# Autodesk Inventor assembly: A2017_T2_01
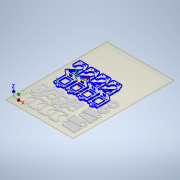
[picture p0: Inventor's stored thumbnail of the model, 180x180]
Saved by Autodesk Inventor 2020 (Build 240168000, 168)
## iProperties
Created: 2021-08-27
Part Number: A2017_T2_01
Document SubType Name: Assembly
Designer: Masato
Author: Masato
## Documents named in this file (8)
- D:\GitHub\inventor\SUSTAINA-OP\Cam\A2017_T2_01.iam
- D:\GitHub\inventor\SUSTAINA-OP\Cam\DisposableBoard.ipt
- D:\GitHub\inventor\SUSTAINA-OP\LowerBody\Ankle\Ankle_back_frame.ipt
- D:\GitHub\inventor\SUSTAINA-OP\LowerBody\Foot\Foot_back_frame.ipt
- D:\GitHub\inventor\SUSTAINA-OP\LowerBody\Foot\Foot_front_frame.ipt
- D:\GitHub\inventor\SUSTAINA-OP\LowerBody\Leg_joit\Leg_joint_pitch_frame.ipt
- D:\GitHub\inventor\SUSTAINA-OP\LowerBody\Ankle\Ankle_side_frame.ipt
- D:\GitHub\inventor\SUSTAINA-OP\UpperBody\Trunk\CrossRollerBearing\Inner_flange.ipt
## Components (19 placed, 7 different names)
1. DisposableBoard:1 — メイト:2, メイト:1, フラッシュ:1, フラッシュ:2, メイト:4, メイト:5, メイト:6, メイト:7, メイト:9, メイト:10, メイト:11, メイト:12, メイト:13, メイト:17, メイト:18, メイト:19, メイト:20, メイト:21, メイト:22, メイト:23, 正接:1, 正接:3, メイト:26, メイト:27, メイト:29, メイト:31, メイト:34, メイト:36, メイト:37, メイト:38, メイト:41, メイト:43, メイト:46, メイト:47, 角度:1, 角度:2
2. Ankle_back_frame:1 — メイト:4, メイト:9, メイト:10, メイト:14, メイト:28, 正接:4
3. Ankle_back_frame:2 — メイト:5, メイト:11, メイト:14, メイト:15
4. Ankle_back_frame:3 — メイト:6, メイト:12, メイト:15, メイト:16, メイト:33, 正接:5
5. Ankle_back_frame:4 — メイト:7, メイト:13, メイト:16
6. Foot_back_frame:2 — メイト:19, メイト:22, メイト:23, メイト:24
7. Foot_front_frame:1 — メイト:17, メイト:21, 正接:2, メイト:25
8. Foot_front_frame:2 — メイト:18, メイト:25, 正接:3, メイト:45, 正接:9
9. Foot_back_frame:3 — メイト:20, 正接:1, メイト:24, 正接:2
10. Leg_joint_pitch_frame:1 — メイト:26, メイト:27, メイト:28, メイト:30, 正接:6
11. Leg_joint_pitch_frame:2 — メイト:31, メイト:32, メイト:33, メイト:35, 正接:7
12. Leg_joint_pitch_frame:3 — メイト:29, メイト:30, 正接:4, メイト:32, メイト:39
13. Leg_joint_pitch_frame:4 — メイト:34, メイト:35, 正接:5
14. Ankle_side_frame:1 — メイト:36, メイト:37, 正接:6, メイト:40
15. Ankle_side_frame:2 — メイト:38, メイト:39, メイト:40, メイト:42
16. Ankle_side_frame:3 — メイト:41, メイト:42, 正接:7, メイト:44
17. Ankle_side_frame:4 — メイト:43, メイト:44, メイト:45, 正接:8, 正接:11
18. Inner_flange:1 — メイト:46, 角度:1, 正接:8, 正接:9, 正接:10
19. Inner_flange:2 — メイト:47, 正接:10, 正接:11, 角度:2
## Relationships (60: Mate 45, Tangent 11, Flush 2, Angle 2)
- メイト:2 [Mate]: DisposableBoard:1
- メイト:1 [Mate]: DisposableBoard:1
- フラッシュ:1 [Flush]: DisposableBoard:1
- フラッシュ:2 [Flush]: DisposableBoard:1
- メイト:4 [Mate]: DisposableBoard:1 ↔ Ankle_back_frame:1
- メイト:5 [Mate]: DisposableBoard:1 ↔ Ankle_back_frame:2
- メイト:6 [Mate]: DisposableBoard:1 ↔ Ankle_back_frame:3
- メイト:7 [Mate]: DisposableBoard:1 ↔ Ankle_back_frame:4
- メイト:9 [Mate] (3 mm): DisposableBoard:1 ↔ Ankle_back_frame:1
- メイト:10 [Mate] (3 mm): DisposableBoard:1 ↔ Ankle_back_frame:1
- メイト:11 [Mate] (3 mm): DisposableBoard:1 ↔ Ankle_back_frame:2
- メイト:12 [Mate] (3 mm): DisposableBoard:1 ↔ Ankle_back_frame:3
- メイト:13 [Mate] (3 mm): DisposableBoard:1 ↔ Ankle_back_frame:4
- メイト:14 [Mate] (2.5 mm): Ankle_back_frame:1 ↔ Ankle_back_frame:2
- メイト:15 [Mate] (2.5 mm): Ankle_back_frame:2 ↔ Ankle_back_frame:3
- メイト:16 [Mate] (2.5 mm): Ankle_back_frame:3 ↔ Ankle_back_frame:4
- メイト:17 [Mate]: DisposableBoard:1 ↔ Foot_front_frame:1
- メイト:18 [Mate]: DisposableBoard:1 ↔ Foot_front_frame:2
- メイト:19 [Mate]: DisposableBoard:1 ↔ Foot_back_frame:2
- メイト:20 [Mate]: DisposableBoard:1 ↔ Foot_back_frame:3
- メイト:21 [Mate] (3 mm): DisposableBoard:1 ↔ Foot_front_frame:1
- メイト:22 [Mate] (3 mm): DisposableBoard:1 ↔ Foot_back_frame:2
- メイト:23 [Mate] (3 mm): DisposableBoard:1 ↔ Foot_back_frame:2
- 正接:1 [Tangent] (3 mm): DisposableBoard:1 ↔ Foot_back_frame:3
- メイト:24 [Mate] (2.5 mm): Foot_back_frame:2 ↔ Foot_back_frame:3
- 正接:2 [Tangent] (2.5 mm): Foot_front_frame:1 ↔ Foot_back_frame:3
- メイト:25 [Mate] (2.5 mm): Foot_front_frame:1 ↔ Foot_front_frame:2
- 正接:3 [Tangent] (3 mm): DisposableBoard:1 ↔ Foot_front_frame:2
- メイト:26 [Mate]: DisposableBoard:1 ↔ Leg_joint_pitch_frame:1
- メイト:27 [Mate] (3 mm): DisposableBoard:1 ↔ Leg_joint_pitch_frame:1
- メイト:28 [Mate] (2.5 mm): Ankle_back_frame:1 ↔ Leg_joint_pitch_frame:1
- メイト:29 [Mate]: DisposableBoard:1 ↔ Leg_joint_pitch_frame:3
- メイト:30 [Mate] (2.5 mm): Leg_joint_pitch_frame:1 ↔ Leg_joint_pitch_frame:3
- 正接:4 [Tangent] (2.5 mm): Ankle_back_frame:1 ↔ Leg_joint_pitch_frame:3
- メイト:31 [Mate]: DisposableBoard:1 ↔ Leg_joint_pitch_frame:2
- メイト:32 [Mate] (2.5 mm): Leg_joint_pitch_frame:2 ↔ Leg_joint_pitch_frame:3
- メイト:33 [Mate] (2.5 mm): Ankle_back_frame:3 ↔ Leg_joint_pitch_frame:2
- メイト:34 [Mate]: DisposableBoard:1 ↔ Leg_joint_pitch_frame:4
- メイト:35 [Mate] (2.5 mm): Leg_joint_pitch_frame:2 ↔ Leg_joint_pitch_frame:4
- 正接:5 [Tangent] (2.5 mm): Ankle_back_frame:3 ↔ Leg_joint_pitch_frame:4
- メイト:36 [Mate]: DisposableBoard:1 ↔ Ankle_side_frame:1
- メイト:37 [Mate] (3 mm): DisposableBoard:1 ↔ Ankle_side_frame:1
- 正接:6 [Tangent] (2.5 mm): Leg_joint_pitch_frame:1 ↔ Ankle_side_frame:1
- メイト:38 [Mate]: DisposableBoard:1 ↔ Ankle_side_frame:2
- メイト:39 [Mate] (2.5 mm): Leg_joint_pitch_frame:3 ↔ Ankle_side_frame:2
- メイト:40 [Mate] (2.5 mm): Ankle_side_frame:1 ↔ Ankle_side_frame:2
- メイト:41 [Mate]: DisposableBoard:1 ↔ Ankle_side_frame:3
- メイト:42 [Mate] (2.5 mm): Ankle_side_frame:2 ↔ Ankle_side_frame:3
- 正接:7 [Tangent] (2.5 mm): Leg_joint_pitch_frame:2 ↔ Ankle_side_frame:3
- メイト:43 [Mate]: DisposableBoard:1 ↔ Ankle_side_frame:4
- メイト:44 [Mate] (2.5 mm): Ankle_side_frame:3 ↔ Ankle_side_frame:4
- メイト:45 [Mate] (2.5 mm): Foot_front_frame:2 ↔ Ankle_side_frame:4
- メイト:46 [Mate]: DisposableBoard:1 ↔ Inner_flange:1
- メイト:47 [Mate]: DisposableBoard:1 ↔ Inner_flange:2
- 角度:1 [Angle] (0 deg): DisposableBoard:1 ↔ Inner_flange:1
- 正接:8 [Tangent] (2.5 mm): Ankle_side_frame:4 ↔ Inner_flange:1
- 正接:9 [Tangent] (2.5 mm): Foot_front_frame:2 ↔ Inner_flange:1
- 正接:10 [Tangent] (2.5 mm): Inner_flange:1 ↔ Inner_flange:2
- 正接:11 [Tangent] (2.5 mm): Ankle_side_frame:4 ↔ Inner_flange:2
- 角度:2 [Angle] (0 deg): DisposableBoard:1 ↔ Inner_flange:2
